# Autodesk Inventor assembly: Jig_assembly
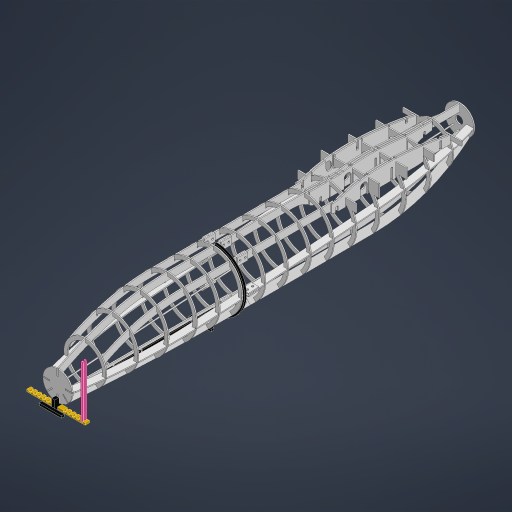
[picture p0: Inventor's stored thumbnail of the model, 512x512]
Saved by Autodesk Inventor 2023 (Build 270158000, 158)
## iProperties
Created: 2023-05-07
Part Number: Jig_assembly
Document SubType Name: Assembly
Designer: szykr
Author: szykr
## Documents named in this file (6)
- D:\Folder Instalacyjny\GitHub Pliki\Solaris\new model\Jig\Jig_assembly.iam
- D:\Folder Instalacyjny\GitHub Pliki\Solaris\new model\nowy kadłub.ipt
- D:\Folder Instalacyjny\GitHub Pliki\Solaris\new model\Jig\Jig_1.ipt
- D:\Folder Instalacyjny\GitHub Pliki\Solaris\new model\Jig\Front_aligner.ipt
- D:\Folder Instalacyjny\GitHub Pliki\Solaris\new model\Jig\Slider.ipt
- D:\Folder Instalacyjny\GitHub Pliki\Solaris\new model\Jig\Widełki.ipt
## Components (5 placed, 5 different names)
1. nowy kadłub:1 — Flush:2
2. Jig_1:1 — Flush:1, Flush:3
3. Front_aligner:1 — Flush:2
4. Slider:1 — Flush:3, Flush:4
5. Widełki:1 — Flush:4
## Relationships (4: Flush 4)
- Flush:1: Jig_1:1
- Flush:2: nowy kadłub:1 ↔ Front_aligner:1
- Flush:3: Jig_1:1 ↔ Slider:1
- Flush:4: Slider:1 ↔ Widełki:1
